# Autodesk Inventor assembly: PruebaIntegracion
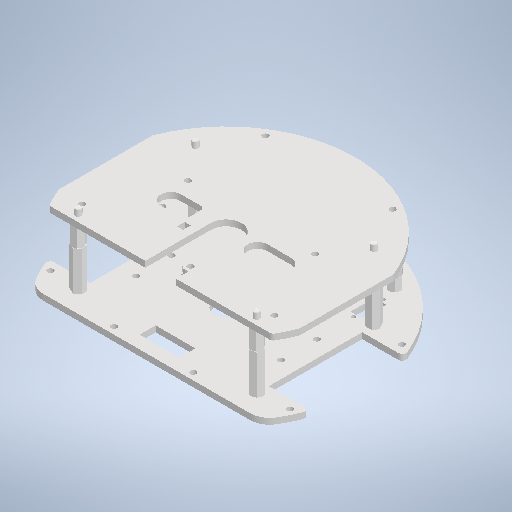
[picture p0: Inventor's stored thumbnail of the model, 512x512]
Saved by Autodesk Inventor 2025.2 (Build 292293000, 293)
## iProperties
Created: 2025-04-23
Part Number: PruebaIntegracion
Document SubType Name: Assembly
Designer: cdavi
Author: cdavi
## Documents named in this file (8)
- D:\Documentos\GIRoM\Atta-Bot-STEM\Chasis\Rediseño_Diego&Carlos\PruebaIntegracion.iam
- D:\Documentos\GIRoM\Atta-Bot-STEM\Chasis\Rediseño_Diego&Carlos\base_chasis_v5\base_chasis_v4-dimsAjustadas.ipt
- D:\Documentos\GIRoM\Atta-Bot-STEM\Chasis\Rediseño_Diego&Carlos\base_chasis_v5.ipt
- D:\Documentos\GIRoM\Atta-Bot-STEM\Chasis\Rediseño_Diego&Carlos\base_nivel2.ipt
- D:\Documentos\GIRoM\Atta-Bot-STEM\Chasis\Rediseño_Diego&Carlos\spacers\hexagonal_spacer_MF_M3_H20_HEX5.5_FTD6_MTL6.ipt
- D:\Documentos\GIRoM\Atta-Bot-STEM\Chasis\Rediseño_Diego&Carlos\spacers\hexagonal_spacer_MF_M3_H10_HEX5.5_FTD6_MTL6.ipt
- D:\Documentos\GIRoM\Atta-Bot-STEM\Chasis\Rediseño_Diego&Carlos\spacers\hexagonal_spacer_MF_M3_H06_HEX5.5_FTD3_MTL6.ipt
- D:\Documentos\GIRoM\Atta-Bot-STEM\Chasis\Rediseño_Diego&Carlos\base_powerboost.ipt
## Components (15 placed, 6 different names)
1. base_chasis_v4-dimsAjustadas:1 — Mate:1, Mate:2, Flush:4, Mate:3, Mate:4, Mate:5, Mate:6, Mate:7, Mate:8, Mate:9, Mate:10, Mate:22, Mate:23, Mate:24, Mate:25, Mate:26, Mate:27, Mate:28, Mate:29
2. base_nivel2:1 — Mate:19, Mate:20, Mate:21
3. hexagonal_spacer_MF_M3_H20_HEX5.5_FTD6_MTL6:1 — Mate:3, Mate:4, Mate:13, Mate:14
4. hexagonal_spacer_MF_M3_H20_HEX5.5_FTD6_MTL6:2 — Mate:5, Mate:6, Mate:11, Mate:12
5. hexagonal_spacer_MF_M3_H20_HEX5.5_FTD6_MTL6:3 — Mate:7, Mate:8, Mate:17, Mate:18
6. hexagonal_spacer_MF_M3_H20_HEX5.5_FTD6_MTL6:4 — Mate:9, Mate:10, Mate:15, Mate:16
7. hexagonal_spacer_MF_M3_H10_HEX5.5_FTD6_MTL6:1 — Mate:11, Mate:12, Mate:19, Mate:21
8. hexagonal_spacer_MF_M3_H10_HEX5.5_FTD6_MTL6:2 — Mate:17, Mate:18
9. hexagonal_spacer_MF_M3_H10_HEX5.5_FTD6_MTL6:3 — Mate:15, Mate:16, Mate:20
10. hexagonal_spacer_MF_M3_H10_HEX5.5_FTD6_MTL6:4 — Mate:13, Mate:14
11. hexagonal_spacer_MF_M3_H06_HEX5.5_FTD3_MTL6:1 — Mate:22, Mate:23, Mate:32, Mate:33
12. hexagonal_spacer_MF_M3_H06_HEX5.5_FTD3_MTL6:2 — Mate:24, Mate:25
13. hexagonal_spacer_MF_M3_H06_HEX5.5_FTD3_MTL6:3 — Mate:26, Mate:27, Mate:30
14. hexagonal_spacer_MF_M3_H06_HEX5.5_FTD3_MTL6:4 — Mate:28, Mate:29
15. base_powerboost:1 — Mate:30, Mate:32, Mate:33
## Relationships (33: Mate 32, Flush 1)
- Mate:1: base_chasis_v4-dimsAjustadas:1
- Mate:2: base_chasis_v4-dimsAjustadas:1
- Flush:4: base_chasis_v4-dimsAjustadas:1
- Mate:3: base_chasis_v4-dimsAjustadas:1 ↔ hexagonal_spacer_MF_M3_H20_HEX5.5_FTD6_MTL6:1
- Mate:4: base_chasis_v4-dimsAjustadas:1 ↔ hexagonal_spacer_MF_M3_H20_HEX5.5_FTD6_MTL6:1
- Mate:5: base_chasis_v4-dimsAjustadas:1 ↔ hexagonal_spacer_MF_M3_H20_HEX5.5_FTD6_MTL6:2
- Mate:6: base_chasis_v4-dimsAjustadas:1 ↔ hexagonal_spacer_MF_M3_H20_HEX5.5_FTD6_MTL6:2
- Mate:7: base_chasis_v4-dimsAjustadas:1 ↔ hexagonal_spacer_MF_M3_H20_HEX5.5_FTD6_MTL6:3
- Mate:8: base_chasis_v4-dimsAjustadas:1 ↔ hexagonal_spacer_MF_M3_H20_HEX5.5_FTD6_MTL6:3
- Mate:9: base_chasis_v4-dimsAjustadas:1 ↔ hexagonal_spacer_MF_M3_H20_HEX5.5_FTD6_MTL6:4
- Mate:10: base_chasis_v4-dimsAjustadas:1 ↔ hexagonal_spacer_MF_M3_H20_HEX5.5_FTD6_MTL6:4
- Mate:11: hexagonal_spacer_MF_M3_H20_HEX5.5_FTD6_MTL6:2 ↔ hexagonal_spacer_MF_M3_H10_HEX5.5_FTD6_MTL6:1
- Mate:12: hexagonal_spacer_MF_M3_H20_HEX5.5_FTD6_MTL6:2 ↔ hexagonal_spacer_MF_M3_H10_HEX5.5_FTD6_MTL6:1
- Mate:13: hexagonal_spacer_MF_M3_H20_HEX5.5_FTD6_MTL6:1 ↔ hexagonal_spacer_MF_M3_H10_HEX5.5_FTD6_MTL6:4
- Mate:14: hexagonal_spacer_MF_M3_H20_HEX5.5_FTD6_MTL6:1 ↔ hexagonal_spacer_MF_M3_H10_HEX5.5_FTD6_MTL6:4
- Mate:15: hexagonal_spacer_MF_M3_H20_HEX5.5_FTD6_MTL6:4 ↔ hexagonal_spacer_MF_M3_H10_HEX5.5_FTD6_MTL6:3
- Mate:16: hexagonal_spacer_MF_M3_H20_HEX5.5_FTD6_MTL6:4 ↔ hexagonal_spacer_MF_M3_H10_HEX5.5_FTD6_MTL6:3
- Mate:17: hexagonal_spacer_MF_M3_H20_HEX5.5_FTD6_MTL6:3 ↔ hexagonal_spacer_MF_M3_H10_HEX5.5_FTD6_MTL6:2
- Mate:18: hexagonal_spacer_MF_M3_H20_HEX5.5_FTD6_MTL6:3 ↔ hexagonal_spacer_MF_M3_H10_HEX5.5_FTD6_MTL6:2
- Mate:19: base_nivel2:1 ↔ hexagonal_spacer_MF_M3_H10_HEX5.5_FTD6_MTL6:1
- Mate:20: base_nivel2:1 ↔ hexagonal_spacer_MF_M3_H10_HEX5.5_FTD6_MTL6:3
- Mate:21: base_nivel2:1 ↔ hexagonal_spacer_MF_M3_H10_HEX5.5_FTD6_MTL6:1
- Mate:22: base_chasis_v4-dimsAjustadas:1 ↔ hexagonal_spacer_MF_M3_H06_HEX5.5_FTD3_MTL6:1
- Mate:23: base_chasis_v4-dimsAjustadas:1 ↔ hexagonal_spacer_MF_M3_H06_HEX5.5_FTD3_MTL6:1
- Mate:24: base_chasis_v4-dimsAjustadas:1 ↔ hexagonal_spacer_MF_M3_H06_HEX5.5_FTD3_MTL6:2
- Mate:25: base_chasis_v4-dimsAjustadas:1 ↔ hexagonal_spacer_MF_M3_H06_HEX5.5_FTD3_MTL6:2
- Mate:26: base_chasis_v4-dimsAjustadas:1 ↔ hexagonal_spacer_MF_M3_H06_HEX5.5_FTD3_MTL6:3
- Mate:27: base_chasis_v4-dimsAjustadas:1 ↔ hexagonal_spacer_MF_M3_H06_HEX5.5_FTD3_MTL6:3
- Mate:28: base_chasis_v4-dimsAjustadas:1 ↔ hexagonal_spacer_MF_M3_H06_HEX5.5_FTD3_MTL6:4
- Mate:29: base_chasis_v4-dimsAjustadas:1 ↔ hexagonal_spacer_MF_M3_H06_HEX5.5_FTD3_MTL6:4
- Mate:30: hexagonal_spacer_MF_M3_H06_HEX5.5_FTD3_MTL6:3 ↔ base_powerboost:1
- Mate:32: hexagonal_spacer_MF_M3_H06_HEX5.5_FTD3_MTL6:1 ↔ base_powerboost:1
- Mate:33: hexagonal_spacer_MF_M3_H06_HEX5.5_FTD3_MTL6:1 ↔ base_powerboost:1
